# Autodesk Inventor assembly: side_mirrored
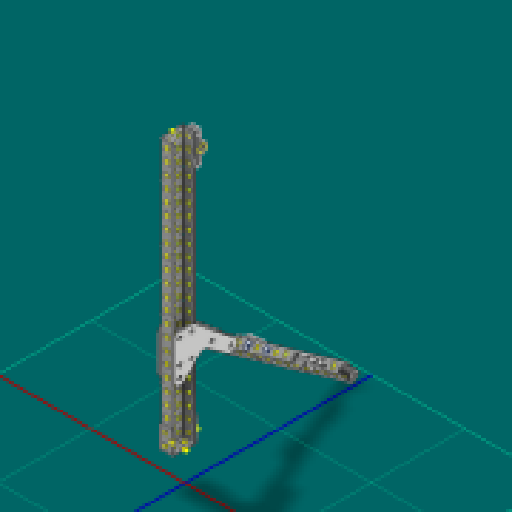
[picture p0: Inventor's stored thumbnail of the model, 512x512]
Saved by Autodesk Inventor 2025 (Build 290162000, 162)
## iProperties
Created: 2024-10-13
Part Number: side_mirrored
Document SubType Name: Assembly
Designer: Averey Ku
Author: Averey Ku
## Documents named in this file (3)
- C:\Users\avere\vex_robotics_high_stakes\hardware\cad\bots\high_stakes_v2\tower\structure\side_mirrored\side_mirrored.iam
- C:\Users\avere\vex_robotics_high_stakes\hardware\cad\bots\high_stakes_v2\tower\structure\side_mirrored\triangle_brace_mirrored.iam
- C:\Users\avere\vex_robotics_high_stakes\hardware\cad\bots\high_stakes_v2\tower\structure\side_mirrored\vertical_mirrored.iam
## Components (2 placed, 2 different names)
1. triangle_brace_mirrored:1 [sub-assembly] — Insert:1, Mate:1
2. vertical_mirrored:1 [sub-assembly] — Insert:1, Mate:1
## Relationships (2: Insert 1, Mate 1)
- Insert:1 (0.5969 mm): triangle_brace_mirrored:1 ↔ vertical_mirrored:1
- Mate:1: triangle_brace_mirrored:1 ↔ vertical_mirrored:1
